# Autodesk Inventor assembly: Assembly1
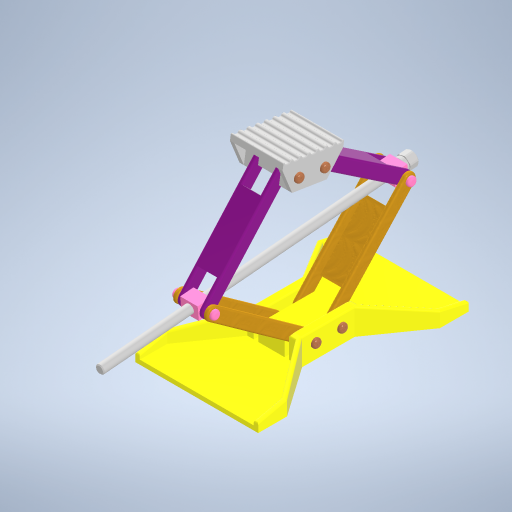
[picture p0: Inventor's stored thumbnail of the model, 512x512]
Saved by Autodesk Inventor 2024 (Build 280153000, 153)
## iProperties
Created: 2024-04-25
Part Number: Assembly1
Document SubType Name: Assembly
Designer: t60147996
Author: t60147996
## Documents named in this file (9)
- E:\Spring 2024\Advanced CAD\Scissor Jack\Assembly1.iam
- E:\Spring 2024\Advanced CAD\Scissor Jack\Base.ipt
- E:\Spring 2024\Advanced CAD\Scissor Jack\Top.ipt
- E:\Spring 2024\Advanced CAD\Scissor Jack\3 Inch Pin.ipt
- E:\Spring 2024\Advanced CAD\Scissor Jack\Insert.ipt
- E:\Spring 2024\Advanced CAD\Scissor Jack\Stopper.ipt
- E:\Spring 2024\Advanced CAD\Scissor Jack\Thick Leg.ipt
- E:\Spring 2024\Advanced CAD\Scissor Jack\Thin Leg.ipt
- E:\Spring 2024\Advanced CAD\Scissor Jack\Through bolt.ipt
## Components (14 placed, 8 different names)
1. Base:1 — Mate:1, Mate:2, Mate:4, Mate:5, Insert:1, Insert:2
2. Top:1 — Mate:6, Insert:5, Insert:8, Insert:9
3. 3 Inch Pin:1 — Mate:1, Mate:2, Mate:3
4. Insert:1 — Insert:6, Mate:7
5. Stopper:1 — Insert:10, Insert:11
6. Thick Leg:1 — Mate:3, Mate:4, Insert:4
7. Thin Leg:1 — Insert:3, Mate:6, Insert:7
8. Through bolt:1 — Insert:10, Mate:7
9. Thick Leg:2 — Mate:5, Insert:2, Insert:3
10. 3 Inch Pin:2 — Insert:1
11. Thin Leg:2 — Insert:4, Insert:5, Insert:6
12. Insert:2 — Insert:7, Insert:11
13. 3 Inch Pin:3 — Insert:8
14. 3 Inch Pin:4 — Insert:9
## Relationships (18: Insert 11, Mate 7)
- Mate:1: Base:1 ↔ 3 Inch Pin:1
- Mate:2: Base:1 ↔ 3 Inch Pin:1
- Mate:3: 3 Inch Pin:1 ↔ Thick Leg:1
- Mate:4: Base:1 ↔ Thick Leg:1
- Mate:5: Base:1 ↔ Thick Leg:2
- Insert:1: Base:1 ↔ 3 Inch Pin:2
- Insert:2: Base:1 ↔ Thick Leg:2
- Insert:3: Thin Leg:1 ↔ Thick Leg:2
- Insert:4: Thick Leg:1 ↔ Thin Leg:2
- Mate:6: Top:1 ↔ Thin Leg:1
- Insert:5: Top:1 ↔ Thin Leg:2
- Insert:6: Insert:1 ↔ Thin Leg:2
- Insert:7: Thin Leg:1 ↔ Insert:2
- Insert:8: Top:1 ↔ 3 Inch Pin:3
- Insert:9: Top:1 ↔ 3 Inch Pin:4
- Insert:10: Stopper:1 ↔ Through bolt:1
- Insert:11: Stopper:1 ↔ Insert:2
- Mate:7: Insert:1 ↔ Through bolt:1
